# Autodesk Inventor assembly: Additional_Building
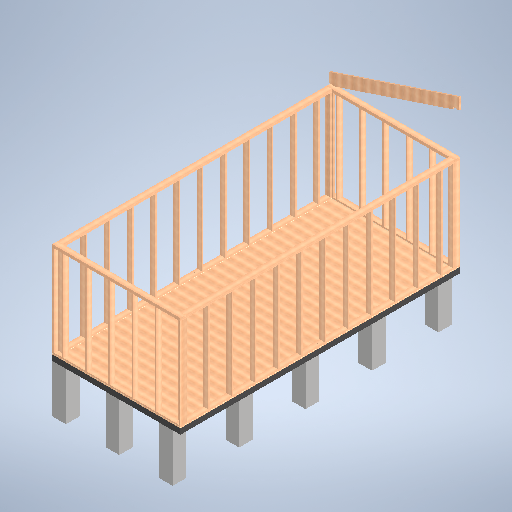
[picture p0: Inventor's stored thumbnail of the model, 512x512]
Saved by Autodesk Inventor 2025 (Build 290162010, 162A)
## iProperties
Created: 2024-08-02
Part Number: Additional_Building
Document SubType Name: Assembly
Designer: Tom
Author: Tom
## Documents named in this file (5)
- C:\Users\Tom\Documents\Inventor\Mobility\Additional_Building\Additional_Building.iam
- C:\Users\Tom\Documents\Inventor\Mobility\Additional_Building\Grid_Of_Piers.iam
- C:\Users\Tom\Documents\Inventor\Mobility\Additional_Building\Floor_System.iam
- C:\Users\Tom\Documents\Inventor\Mobility\Additional_Building\Walls.iam
- C:\Users\Tom\Documents\Inventor\Mobility\Additional_Building\Rafter.ipt
## Components (4 placed, 4 different names)
1. Grid_Of_Piers:1 [sub-assembly] — Mate:12, Mate:13, Flush:7
2. Floor_System:1 [sub-assembly] — Mate:12, Mate:13, Flush:7, Mate:14, Flush:8, Flush:9
3. Walls:1 [sub-assembly] — Mate:14, Flush:8, Flush:9, Mate:15, Flush:10, Mate:16
4. Rafter:1 — Mate:15, Flush:10, Mate:16
## Relationships (9: Mate 5, Flush 4)
- Mate:12: Grid_Of_Piers:1 ↔ Floor_System:1
- Mate:13: Grid_Of_Piers:1 ↔ Floor_System:1
- Flush:7: Grid_Of_Piers:1 ↔ Floor_System:1
- Mate:14: Floor_System:1 ↔ Walls:1
- Flush:8: Floor_System:1 ↔ Walls:1
- Flush:9: Floor_System:1 ↔ Walls:1
- Mate:15: Walls:1 ↔ Rafter:1
- Flush:10: Walls:1 ↔ Rafter:1
- Mate:16: Walls:1 ↔ Rafter:1
